# Autodesk Inventor assembly: UBG-Rad
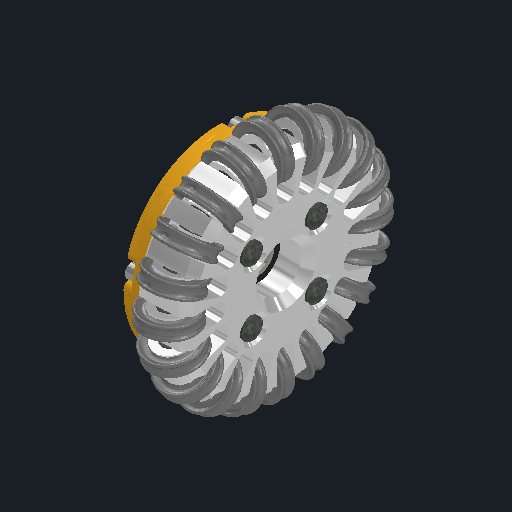
[picture p0: Inventor's stored thumbnail of the model, 512x512]
Saved by Autodesk Inventor 2025.2 (Build 292293000, 293)
## iProperties
Created: 2024-11-07
Part Number: UBG-Rad
Document SubType Name: Assembly
Designer: Fabian
Author: Fabian
## Documents named in this file (9)
- C:\Users\Faabs\Desktop\HBG v2025\Unterbaugruppen\UBG-Rad\UBG-Rad.iam
- C:\Users\Faabs\Desktop\HBG v2025\Unterbaugruppen\UBG-Rad\Bauteile\Radkörper\60z.ipt
- C:\Users\Faabs\Desktop\HBG v2025\Unterbaugruppen\UBG-Rad\Bauteile\Radkörper\Raddeckel.ipt
- C:\Users\Faabs\Desktop\HBG v2025\Unterbaugruppen\UBG-Rad\Bauteile\Radkörper\Radkasten.ipt
- C:\Users\Faabs\Desktop\HBG v2025\Unterbaugruppen\UBG-Rad\Bauteile\Rolle\UBG-Rolle.iam
- C:\Users\Faabs\Desktop\HBG v2025\Verbindungselemente\ISO 10642\ISO 10642  - M3  x  8.ipt
- C:\Users\Faabs\Desktop\HBG v2025\Verbindungselemente\DIN 912\DIN 912 - M2 x 0,4 x 6 x 5.ipt
- C:\Users\Faabs\Desktop\HBG v2025\Unterbaugruppen\UBG-Rad\Bauteile\Radkörper\Kugellager 14 x 7 x 5.ipt
- Kugellager 17 x 7 x 5.ipt
## Components (32 placed, 7 different names)
1. 60z:1 — Fluchtend:1, Passend:1, Passend:2, Passend:3, Passend:4, Passend:5, Einfügen:5, Einfügen:6, Einfügen:7, Einfügen:8
2. Raddeckel:1 — Passend:9, Passend:10, Passend:11, Einfügen:1, Einfügen:2, Einfügen:3, Einfügen:4
3. Radkasten:1 — Passend:3, Passend:4, Passend:5, Winkel:1, Passend:6, Passend:7, Passend:8, Passend:9, Passend:10, Passend:11, Passend:12, Passend:13
4. Kugellager 17 x 7 x 5:1 — Passend:12, Passend:13
5. DIN EN ISO 10642 M3  x  8:1 — Einfügen:2
6. DIN EN ISO 10642 M3  x  8:2 — Einfügen:3
7. DIN EN ISO 10642 M3  x  8:3 — Einfügen:1
8. DIN EN ISO 10642 M3  x  8:4 — Einfügen:4
9. DIN 912 - ersetzt durch DIN EN ISO 4762 M2 x 6:1 — Einfügen:7
10. DIN 912 - ersetzt durch DIN EN ISO 4762 M2 x 6:2 — Einfügen:8
11. DIN 912 - ersetzt durch DIN EN ISO 4762 M2 x 6:3 — Einfügen:6
12. DIN 912 - ersetzt durch DIN EN ISO 4762 M2 x 6:4 — Einfügen:5
13. UBG-Rolle:1 [sub-assembly] — Passend:6, Passend:7, Passend:8
14. UBG-Rolle:2 [sub-assembly]
15. UBG-Rolle:3 [sub-assembly]
16. UBG-Rolle:4 [sub-assembly]
17. UBG-Rolle:5 [sub-assembly]
18. UBG-Rolle:6 [sub-assembly]
19. UBG-Rolle:7 [sub-assembly]
20. UBG-Rolle:8 [sub-assembly]
21. UBG-Rolle:9 [sub-assembly]
22. UBG-Rolle:10 [sub-assembly]
23. UBG-Rolle:11 [sub-assembly]
24. UBG-Rolle:12 [sub-assembly]
25. UBG-Rolle:13 [sub-assembly]
26. UBG-Rolle:14 [sub-assembly]
27. UBG-Rolle:15 [sub-assembly]
28. UBG-Rolle:16 [sub-assembly]
29. UBG-Rolle:17 [sub-assembly]
30. UBG-Rolle:18 [sub-assembly]
31. UBG-Rolle:19 [sub-assembly]
32. UBG-Rolle:20 [sub-assembly]
## Component patterns: (20 elements, first: UBG-Rolle:1)
## Relationships (23: Mate 13, Insert 8, Flush 1, Angle 1)
- Fluchtend:1 [Flush]: 60z:1
- Passend:1 [Mate]: 60z:1
- Passend:2 [Mate]: 60z:1
- Passend:3 [Mate]: 60z:1 ↔ Radkasten:1
- Passend:4 [Mate]: 60z:1 ↔ Radkasten:1
- Passend:5 [Mate]: 60z:1 ↔ Radkasten:1
- Winkel:1 [Angle] (0 deg): Radkasten:1
- Passend:6 [Mate] (0.1 mm): Radkasten:1 ↔ UBG-Rolle:1
- Passend:7 [Mate]: Radkasten:1 ↔ UBG-Rolle:1
- Passend:8 [Mate] (0.025 mm): Radkasten:1 ↔ UBG-Rolle:1
- Passend:9 [Mate]: Raddeckel:1 ↔ Radkasten:1
- Passend:10 [Mate]: Raddeckel:1 ↔ Radkasten:1
- Passend:11 [Mate]: Raddeckel:1 ↔ Radkasten:1
- Einfügen:1 [Insert]: Raddeckel:1 ↔ DIN EN ISO 10642 M3  x  8:3
- Einfügen:2 [Insert]: Raddeckel:1 ↔ DIN EN ISO 10642 M3  x  8:1
- Einfügen:3 [Insert]: Raddeckel:1 ↔ DIN EN ISO 10642 M3  x  8:2
- Einfügen:4 [Insert]: Raddeckel:1 ↔ DIN EN ISO 10642 M3  x  8:4
- Einfügen:5 [Insert]: 60z:1 ↔ DIN 912 - ersetzt durch DIN EN ISO 4762 M2 x 6:4
- Einfügen:6 [Insert]: 60z:1 ↔ DIN 912 - ersetzt durch DIN EN ISO 4762 M2 x 6:3
- Einfügen:7 [Insert]: 60z:1 ↔ DIN 912 - ersetzt durch DIN EN ISO 4762 M2 x 6:1
- Einfügen:8 [Insert]: 60z:1 ↔ DIN 912 - ersetzt durch DIN EN ISO 4762 M2 x 6:2
- Passend:12 [Mate]: Radkasten:1 ↔ Kugellager 17 x 7 x 5:1
- Passend:13 [Mate]: Radkasten:1 ↔ Kugellager 17 x 7 x 5:1
